# Autodesk Inventor assembly: ROV
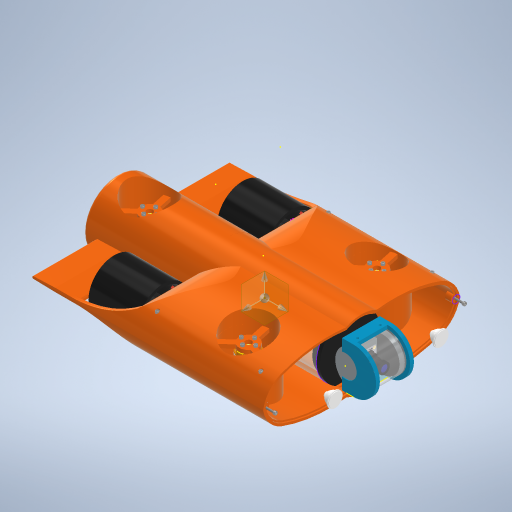
[picture p0: Inventor's stored thumbnail of the model, 512x512]
Saved by Autodesk Inventor 2024 (Build 280153000, 153)
## iProperties
Created: 2025-05-20
Part Number: ROV
Document SubType Name: Assembly
Designer: Paweł
Mass: 2542.62 g
Surface Area: 7080.55 cm^2
Volume: 2465.84 cm^3
Density: 1.03114 g/cm^3
Author: Paweł
## Documents named in this file (22)
- F:\ROV\ROV.iam
- F:\ROV\PROP.ipt
- F:\ROV\silnik.ipt
- F:\ROV\tuba.ipt
- F:\ROV\pokrywka.ipt
- F:\ROV\camera_pipe.ipt
- F:\ROV\camera_poprywka.ipt
- F:\ROV\przód.ipt
- F:\ROV\przód2.ipt
- F:\ROV\korpus3.ipt
- F:\ROV\TIR_lens_12.8mm.ipt
- C:\Users\Paweł\OneDrive\Dokumenty\Inventor\Content Center Files\R2024\pl-PL\ISO 4762(2)\ISO 4762 - M2,5 x 20ISO.ipt
- F:\ROV\korpus3_gora.ipt
- F:\ROV\osłonasilnik.ipt
- F:\ROV\1000KV Brushless Motor.ipt
- C:\Users\Paweł\OneDrive\Dokumenty\Inventor\Content Center Files\R2024\pl-PL\ISO 4036(1)\ISO 4036 - M4(1).ipt
- C:\Users\Paweł\OneDrive - Politechnika Warszawska\PROJEKTOWANIE ROBOTÓW\propellersmall.ipt
- F:\ROV\PROP 2.ipt
- C:\Users\Paweł\OneDrive\Dokumenty\Inventor\Content Center Files\R2024\pl-PL\DIN EN 24 036(2)\DIN EN 24 036 - M3.ipt
- C:\Users\Paweł\OneDrive\Dokumenty\Inventor\Content Center Files\R2024\pl-PL\ISO 4762(1)\DIN EN ISO 4762 - M2,5 x 4.ipt
- F:\ROV\Camera Module Assem\Camera Module Assem.iam
- F:\ROV\camera_poprywka_bez mocowania.ipt
## Components (61 placed, 21 different names)
1. PROP:1 — Wstawiające:16, Wstawiające:33
2. silnik:1 — Zestawiające:21, Wstawiające:16, Wstawiające:24, Wstawiające:25
3. tuba:1 — Wstawiające:3, Wstawiające:4, Styczny:1
4. pokrywka:1 — Wstawiające:3, Równoległe:1
5. pokrywka:2 — Wstawiające:4
6. camera_pipe:1 — Wstawiające:58, Wstawiające:60
7. przód:1 — Zestawiające:9, Zestawiające:10, Równoległe:2, Równoległe:3, Zestawiające:14, Zestawiające:15, Wstawiające:32, Wstawiające:62
8. przód2:1 — Zestawiające:14, Zestawiające:15, Wstawiające:61
9. korpus3:1 — Równoległe:1, Styczny:1, Zestawiające:21, Wstawiające:18, Wstawiające:19, Wstawiające:20, Wstawiające:21, Wstawiające:22, Wstawiające:23, Wstawiające:24, Wstawiające:25, Wstawiające:26, Zestawiające:23, Zestawiające:24, Zestawiające:25, Wstawiające:29, Wstawiające:31, Wstawiające:32, Wstawiające:41, Wstawiające:42, Wstawiające:43, Wstawiające:44, Wstawiające:45, Wstawiające:46, Wstawiające:47, Wstawiające:48, Wstawiające:49, Wstawiające:50, Wstawiające:51, Wstawiające:52, Wstawiające:62, Wstawiające:63, Wstawiające:64, Wstawiające:65, Wstawiające:66, Wstawiające:67, Wstawiające:68, Wstawiające:69, Wstawiające:70, Wstawiające:71, Wstawiające:72, Wstawiające:73, Wstawiające:74, Wstawiające:75, Wstawiające:76
10. TIR_lens_12.8mm:1 — Zestawiające:9, Równoległe:3
11. TIR_lens_12.8mm:2 — Zestawiające:10, Równoległe:2
12. ISO 4762 M2,5 x 20:1
13. ISO 4762 M2,5 x 20:2
14. korpus3_gora:1 — Wstawiające:54, Wstawiające:55, Wstawiające:56, Wstawiające:57, Wstawiające:63, Wstawiające:64
15. PROP:2 — Wstawiające:34
16. silnik:2 — Wstawiające:18, Wstawiające:19
17. osłonasilnik:1 — Wstawiające:20, Wstawiające:21
18. osłonasilnik:2 — Wstawiające:22, Wstawiające:23
19. 1000KV Brushless Motor:1 — Wstawiające:29, Wstawiające:37
20. 1000KV Brushless Motor:2 — Wstawiające:26, Wstawiające:36
21. 1000KV Brushless Motor:3 — Wstawiające:31, Wstawiające:35
22. DIN EN 24036 M4:1 — Wstawiające:33
23. DIN EN 24036 M4:2 — Wstawiające:34
24. propellersmall:1
25. PROP 2:1 — Wstawiające:36, Wstawiające:39
26. PROP 2:2 — Wstawiające:37, Wstawiające:38
27. PROP 2:3 — Wstawiające:35, Wstawiające:40
28. DIN EN 24036 M3:1 — Wstawiające:38
29. DIN EN 24036 M3:2 — Wstawiające:39
30. DIN EN 24036 M3:3 — Wstawiające:40
31. DIN EN ISO 4762 M2,5 x 4:1 — Wstawiające:41
32. DIN EN ISO 4762 M2,5 x 4:2 — Wstawiające:42
33. DIN EN ISO 4762 M2,5 x 4:3 — Wstawiające:43
34. DIN EN ISO 4762 M2,5 x 4:4 — Wstawiające:44
35. DIN EN ISO 4762 M2,5 x 4:5 — Wstawiające:45
36. DIN EN ISO 4762 M2,5 x 4:6 — Wstawiające:46
37. DIN EN ISO 4762 M2,5 x 4:7 — Wstawiające:47
38. DIN EN ISO 4762 M2,5 x 4:8 — Wstawiające:48
39. DIN EN ISO 4762 M2,5 x 4:9 — Wstawiające:49
40. DIN EN ISO 4762 M2,5 x 4:10 — Wstawiające:50
41. DIN EN ISO 4762 M2,5 x 4:11 — Wstawiające:51
42. DIN EN ISO 4762 M2,5 x 4:12 — Wstawiające:52
43. DIN EN ISO 4762 M2,5 x 4:13 — Wstawiające:54
44. DIN EN ISO 4762 M2,5 x 4:14 — Wstawiające:55
45. DIN EN ISO 4762 M2,5 x 4:15 — Wstawiające:56
46. DIN EN ISO 4762 M2,5 x 4:16 — Wstawiające:57
47. Camera Module Assem:1 [sub-assembly] — Wstawiające:59, Zestawiające:26
48. camera_poprywka:1 — Wstawiające:59, Zestawiające:26, Wstawiające:60
49. camera_poprywka_bez mocowania:1 — Wstawiające:58, Wstawiające:61
50. DIN EN ISO 4762 M2,5 x 4:17 — Wstawiające:65
51. DIN EN ISO 4762 M2,5 x 4:18 — Wstawiające:66
52. DIN EN ISO 4762 M2,5 x 4:19 — Wstawiające:67
53. DIN EN ISO 4762 M2,5 x 4:20 — Wstawiające:68
54. DIN EN ISO 4762 M2,5 x 4:21 — Wstawiające:69
55. DIN EN ISO 4762 M2,5 x 4:22 — Wstawiające:70
56. DIN EN ISO 4762 M2,5 x 4:23 — Wstawiające:71
57. DIN EN ISO 4762 M2,5 x 4:24 — Wstawiające:72
58. DIN EN ISO 4762 M2,5 x 4:25 — Wstawiające:73
59. DIN EN ISO 4762 M2,5 x 4:26 — Wstawiające:74
60. DIN EN ISO 4762 M2,5 x 4:27 — Wstawiające:75
61. DIN EN ISO 4762 M2,5 x 4:28 — Wstawiające:76
## Relationships (72: Insert 59, Mate 9, Flush 3, Tangent 1)
- Wstawiające:3 [Insert]: tuba:1 ↔ pokrywka:1
- Wstawiające:4 [Insert]: tuba:1 ↔ pokrywka:2
- Równoległe:1 [Flush] (15 mm): pokrywka:1 ↔ korpus3:1
- Styczny:1 [Tangent]: tuba:1 ↔ korpus3:1
- Zestawiające:9 [Mate]: przód:1 ↔ TIR_lens_12.8mm:1
- Zestawiające:10 [Mate]: przód:1 ↔ TIR_lens_12.8mm:2
- Równoległe:2 [Flush]: przód:1 ↔ TIR_lens_12.8mm:2
- Równoległe:3 [Flush]: przód:1 ↔ TIR_lens_12.8mm:1
- Zestawiające:14 [Mate]: przód:1 ↔ przód2:1
- Zestawiające:15 [Mate]: przód:1 ↔ przód2:1
- Zestawiające:21 [Mate]: silnik:1 ↔ korpus3:1
- Wstawiające:16 [Insert]: PROP:1 ↔ silnik:1
- [Insert]: PROP:2 ↔ silnik:2
- Wstawiające:18 [Insert]: korpus3:1 ↔ silnik:2
- Wstawiające:19 [Insert]: korpus3:1 ↔ silnik:2
- Wstawiające:20 [Insert]: korpus3:1 ↔ osłonasilnik:1
- Wstawiające:21 [Insert]: korpus3:1 ↔ osłonasilnik:1
- Wstawiające:22 [Insert]: korpus3:1 ↔ osłonasilnik:2
- Wstawiające:23 [Insert]: korpus3:1 ↔ osłonasilnik:2
- Wstawiające:24 [Insert]: silnik:1 ↔ korpus3:1
- Wstawiające:25 [Insert]: silnik:1 ↔ korpus3:1
- Wstawiające:26 [Insert]: korpus3:1 ↔ 1000KV Brushless Motor:2
- Zestawiające:23 [Mate]: korpus3:1
- Zestawiające:24 [Mate]: korpus3:1
- Zestawiające:25 [Mate]: korpus3:1
- Wstawiające:29 [Insert]: korpus3:1 ↔ 1000KV Brushless Motor:1
- Wstawiające:31 [Insert]: korpus3:1 ↔ 1000KV Brushless Motor:3
- Wstawiające:32 [Insert]: przód:1 ↔ korpus3:1
- Wstawiające:33 [Insert]: PROP:1 ↔ DIN EN 24036 M4:1
- Wstawiające:34 [Insert]: PROP:2 ↔ DIN EN 24036 M4:2
- Wstawiające:35 [Insert]: 1000KV Brushless Motor:3 ↔ PROP 2:3
- Wstawiające:36 [Insert]: 1000KV Brushless Motor:2 ↔ PROP 2:1
- Wstawiające:37 [Insert]: 1000KV Brushless Motor:1 ↔ PROP 2:2
- Wstawiające:38 [Insert]: PROP 2:2 ↔ DIN EN 24036 M3:1
- Wstawiające:39 [Insert]: PROP 2:1 ↔ DIN EN 24036 M3:2
- Wstawiające:40 [Insert]: PROP 2:3 ↔ DIN EN 24036 M3:3
- Wstawiające:41 [Insert]: korpus3:1 ↔ DIN EN ISO 4762 M2,5 x 4:1
- Wstawiające:42 [Insert]: korpus3:1 ↔ DIN EN ISO 4762 M2,5 x 4:2
- Wstawiające:43 [Insert]: korpus3:1 ↔ DIN EN ISO 4762 M2,5 x 4:3
- Wstawiające:44 [Insert]: korpus3:1 ↔ DIN EN ISO 4762 M2,5 x 4:4
- Wstawiające:45 [Insert]: korpus3:1 ↔ DIN EN ISO 4762 M2,5 x 4:5
- Wstawiające:46 [Insert]: korpus3:1 ↔ DIN EN ISO 4762 M2,5 x 4:6
- Wstawiające:47 [Insert]: korpus3:1 ↔ DIN EN ISO 4762 M2,5 x 4:7
- Wstawiające:48 [Insert]: korpus3:1 ↔ DIN EN ISO 4762 M2,5 x 4:8
- Wstawiające:49 [Insert]: korpus3:1 ↔ DIN EN ISO 4762 M2,5 x 4:9
- Wstawiające:50 [Insert]: korpus3:1 ↔ DIN EN ISO 4762 M2,5 x 4:10
- Wstawiające:51 [Insert]: korpus3:1 ↔ DIN EN ISO 4762 M2,5 x 4:11
- Wstawiające:52 [Insert]: korpus3:1 ↔ DIN EN ISO 4762 M2,5 x 4:12
- Wstawiające:54 [Insert]: korpus3_gora:1 ↔ DIN EN ISO 4762 M2,5 x 4:13
- Wstawiające:55 [Insert]: korpus3_gora:1 ↔ DIN EN ISO 4762 M2,5 x 4:14
- Wstawiające:56 [Insert]: korpus3_gora:1 ↔ DIN EN ISO 4762 M2,5 x 4:15
- Wstawiające:57 [Insert]: korpus3_gora:1 ↔ DIN EN ISO 4762 M2,5 x 4:16
- Wstawiające:58 [Insert]: camera_pipe:1 ↔ camera_poprywka_bez mocowania:1
- Wstawiające:59 [Insert]: Camera Module Assem:1 ↔ camera_poprywka:1
- Zestawiające:26 [Mate]: Camera Module Assem:1 ↔ camera_poprywka:1
- Wstawiające:60 [Insert]: camera_pipe:1 ↔ camera_poprywka:1
- Wstawiające:61 [Insert]: przód2:1 ↔ camera_poprywka_bez mocowania:1
- Wstawiające:62 [Insert]: przód:1 ↔ korpus3:1
- Wstawiające:63 [Insert]: korpus3:1 ↔ korpus3_gora:1
- Wstawiające:64 [Insert]: korpus3:1 ↔ korpus3_gora:1
- Wstawiające:65 [Insert]: korpus3:1 ↔ DIN EN ISO 4762 M2,5 x 4:17
- Wstawiające:66 [Insert]: korpus3:1 ↔ DIN EN ISO 4762 M2,5 x 4:18
- Wstawiające:67 [Insert]: korpus3:1 ↔ DIN EN ISO 4762 M2,5 x 4:19
- Wstawiające:68 [Insert]: korpus3:1 ↔ DIN EN ISO 4762 M2,5 x 4:20
- Wstawiające:69 [Insert]: korpus3:1 ↔ DIN EN ISO 4762 M2,5 x 4:21
- Wstawiające:70 [Insert]: korpus3:1 ↔ DIN EN ISO 4762 M2,5 x 4:22
- Wstawiające:71 [Insert]: korpus3:1 ↔ DIN EN ISO 4762 M2,5 x 4:23
- Wstawiające:72 [Insert]: korpus3:1 ↔ DIN EN ISO 4762 M2,5 x 4:24
- Wstawiające:73 [Insert]: korpus3:1 ↔ DIN EN ISO 4762 M2,5 x 4:25
- Wstawiające:74 [Insert]: korpus3:1 ↔ DIN EN ISO 4762 M2,5 x 4:26
- Wstawiające:75 [Insert]: korpus3:1 ↔ DIN EN ISO 4762 M2,5 x 4:27
- Wstawiające:76 [Insert]: korpus3:1 ↔ DIN EN ISO 4762 M2,5 x 4:28
## Named parameters: d84_d83 = 0 mm
